# Autodesk Inventor assembly: Arm_Left
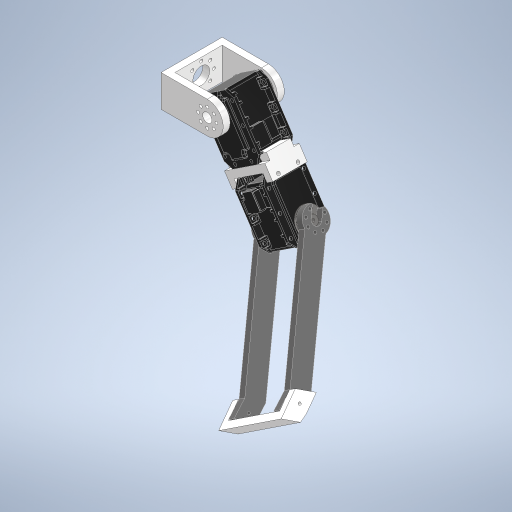
[picture p0: Inventor's stored thumbnail of the model, 512x512]
Saved by Autodesk Inventor 2024.3 (Build 283343000, 343)
## iProperties
Created: 2024-09-18
Part Number: Arm_Left
Document SubType Name: Assembly
Designer: 구지현
Author: 구지현
## Documents named in this file (8)
- C:\Users\구지현\Desktop\19th_intern_kdy_fight_robot\부품\Upper_Body\Arm\Arm_Left.iam
- C:\Users\구지현\Desktop\19th_intern_kdy_fight_robot\부품\Upper_Body\Arm\Hand_Connection_Parts.ipt
- C:\Users\구지현\Desktop\19th_intern_kdy_fight_robot\부품\Upper_Body\Arm\Middle_Arm_Fixing_Parts.ipt
- C:\Users\구지현\Desktop\19th_intern_kdy_fight_robot\부품\Upper_Body\Arm\Shoulder_Fixing_Parts_Left.ipt
- C:\Users\구지현\Desktop\19th_intern_kdy_fight_robot\부품\Upper_Body\Arm\Hand.ipt
- C:\Users\구지현\Desktop\19th_intern_kdy_fight_robot\부품\ROBOTIS(Inventor 2024 ver.)\다이나믹셀\MX-28T_R+idle.ipt.iam
- C:\Users\구지현\Desktop\19th_intern_kdy_fight_robot\부품\ROBOTIS(Inventor 2024 ver.)\혼\28Horn.ipt
- MX-28T_R+idle.ipt
## Components (8 placed, 6 different names)
1. Hand:1 — 삽입:10, 메이트:3, 메이트:4, 메이트:5
2. Hand_Connection_Parts:1 — 삽입:10
3. Middle_Arm_Fixing_Parts:1 — 메이트:1, 메이트:2, 메이트:6, 메이트:7
4. Shoulder_Fixing_Parts_Left:1 — 삽입:13
5. MX-28T_R+idle.ipt:1 [sub-assembly] — 삽입:12, 메이트:5, 메이트:6, 메이트:7
6. 28Horn:1 — 삽입:11, 삽입:13
7. MX-28T_R+idle.ipt:2 [sub-assembly] — 삽입:11, 메이트:1, 메이트:2
8. 28Horn:2 — 삽입:12, 메이트:3, 메이트:4
## Relationships (11: Mate 7, Insert 4)
- 삽입:10 [Insert]: Hand:1 ↔ Hand_Connection_Parts:1
- 삽입:11 [Insert]: 28Horn:1 ↔ MX-28T_R+idle.ipt:2
- 삽입:12 [Insert]: MX-28T_R+idle.ipt:1 ↔ 28Horn:2
- 삽입:13 [Insert]: Shoulder_Fixing_Parts_Left:1 ↔ 28Horn:1
- 메이트:1 [Mate]: Middle_Arm_Fixing_Parts:1 ↔ MX-28T_R+idle.ipt:2
- 메이트:2 [Mate]: Middle_Arm_Fixing_Parts:1 ↔ MX-28T_R+idle.ipt:2
- 메이트:3 [Mate]: Hand:1 ↔ 28Horn:2
- 메이트:4 [Mate]: Hand:1 ↔ 28Horn:2
- 메이트:5 [Mate]: Hand:1 ↔ MX-28T_R+idle.ipt:1
- 메이트:6 [Mate]: Middle_Arm_Fixing_Parts:1 ↔ MX-28T_R+idle.ipt:1
- 메이트:7 [Mate]: Middle_Arm_Fixing_Parts:1 ↔ MX-28T_R+idle.ipt:1
